# Autodesk Inventor assembly: LeadScrewArrangement
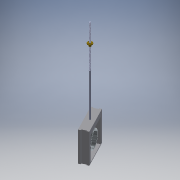
[picture p0: Inventor's stored thumbnail of the model, 180x180]
Saved by Autodesk Inventor 2019 (Build 230136000, 136)
## iProperties
Created: 2019-06-28
Part Number: LeadScrewArrangement
Document SubType Name: Assembly
Designer: dell
Author: dell
## Documents named in this file (5)
- C:\Users\Satwik Pandey\Desktop\RuTAG Project\New folder\LeadScrewArrangement.iam
- C:\Users\Satwik Pandey\Desktop\RuTAG Project\New folder\LeadScrewBox.ipt
- C:\Users\Satwik Pandey\Desktop\RuTAG Project\New folder\LeadScrew.ipt
- C:\Users\Satwik Pandey\Desktop\RuTAG Project\New folder\LeadScrewNut.ipt
- C:\Users\Satwik Pandey\Desktop\RuTAG Project\New folder\project flange bearing part1_MIR7_MIR.ipt
## Components (4 placed, 4 different names)
1. LeadScrewBox:1 — Flush:1, Mate:6, Mate:9, Mate:10, Mate:11
2. LeadScrew:1 — Mate:6, Mate:7, Mate:8
3. LeadScrewNut:1 — Mate:8
4. project flange bearing part1_MIR7_MIR:1 — Mate:9, Mate:10, Mate:11
## Relationships (10: Mate 9, Flush 1)
- Flush:1 (-20 mm): LeadScrewBox:1
- Mate:3
- Mate:4
- Mate:5
- Mate:6: LeadScrewBox:1 ↔ LeadScrew:1
- Mate:7: LeadScrew:1
- Mate:8: LeadScrew:1 ↔ LeadScrewNut:1
- Mate:9: LeadScrewBox:1 ↔ project flange bearing part1_MIR7_MIR:1
- Mate:10: LeadScrewBox:1 ↔ project flange bearing part1_MIR7_MIR:1
- Mate:11: LeadScrewBox:1 ↔ project flange bearing part1_MIR7_MIR:1
